# Autodesk Inventor assembly: Shooter Assembly
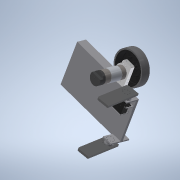
[picture p0: Inventor's stored thumbnail of the model, 180x180]
Saved by Autodesk Inventor 2021 (Build 250183000, 183)
## iProperties
Created: 2020-10-17
Part Number: Shooter Assembly
Document SubType Name: Assembly
Designer: Delta
Author: Delta
## Documents named in this file (9)
- C:\Robotics\CAD\2020-21-CAD\Shooter\Shooter Assembly.iam
- C:\Robotics\CAD\2020-21-CAD\Shooter\Guide.ipt
- C:\Robotics\CAD\2020-21-CAD\Shooter\Axle Rotate.ipt
- C:\Robotics\CAD\2020-21-CAD\Shooter\Triangle axle slide connector.ipt
- C:\Robotics\CAD\2020-21-CAD\Shooter\Tetrex 2pc motor mount.ipt
- C:\Robotics\CAD\2020-21-CAD\Shooter\motor-3102NeveRest20 (1).ipt
- C:\Robotics\CAD\2020-21-CAD\Shooter\Flywheel_4inWheel8mmHub.ipt
- C:\Robotics\CAD\2020-21-CAD\Shooter\Tetrix bracket - single servo.ipt
- C:\Robotics\CAD\COTSParts\Rev\REV-41-1097SmartServo.ipt
## Components (10 placed, 8 different names)
1. Guide:1 — Mate:14, Mate:15, Angle:1, Angle:2, Mate:37, Mate:38, Mate:39, Mate:40, Mate:43, Flush:8, Mate:44
2. Axle Rotate:1 — Mate:9, Mate:13, Mate:40
3. Axle Rotate:2 — Mate:8, Mate:12, Mate:37, Mate:38, Mate:39
4. Triangle axle slide connector:1 — Mate:8, Mate:12, Flush:9, Flush:10
5. Triangle axle slide connector:2 — Mate:9, Mate:13, Flush:9, Flush:10
6. Tetrex 2pc motor mount:1 — Mate:14, Mate:15, Angle:1, Mate:16, Mate:17
7. motor-3102NeveRest20 (1):1 — Mate:16, Mate:17, Mate:18, Mate:19, Angle:2
8. Flywheel_4inWheel8mmHub:1 — Mate:18, Mate:19
9. Tetrix bracket - single servo:1 — Mate:25, Mate:41, Mate:42, Mate:43, Flush:8
10. REV-41-1097SmartServo:1 — Mate:25, Mate:41, Mate:42, Mate:44
## Relationships (24: Mate 19, Flush 3, Angle 2)
- Mate:8: Axle Rotate:2 ↔ Triangle axle slide connector:1
- Mate:9: Axle Rotate:1 ↔ Triangle axle slide connector:2
- Mate:12: Axle Rotate:2 ↔ Triangle axle slide connector:1
- Mate:13: Axle Rotate:1 ↔ Triangle axle slide connector:2
- Mate:14: Guide:1 ↔ Tetrex 2pc motor mount:1
- Mate:15: Guide:1 ↔ Tetrex 2pc motor mount:1
- Angle:1 (0 deg): Guide:1 ↔ Tetrex 2pc motor mount:1
- Mate:16: Tetrex 2pc motor mount:1 ↔ motor-3102NeveRest20 (1):1
- Mate:17: Tetrex 2pc motor mount:1 ↔ motor-3102NeveRest20 (1):1
- Mate:18: motor-3102NeveRest20 (1):1 ↔ Flywheel_4inWheel8mmHub:1
- Mate:19: motor-3102NeveRest20 (1):1 ↔ Flywheel_4inWheel8mmHub:1
- Angle:2 (0 deg): Guide:1 ↔ motor-3102NeveRest20 (1):1
- Mate:25: Tetrix bracket - single servo:1 ↔ REV-41-1097SmartServo:1
- Mate:37: Guide:1 ↔ Axle Rotate:2
- Mate:38: Guide:1 ↔ Axle Rotate:2
- Mate:39: Guide:1 ↔ Axle Rotate:2
- Mate:40: Guide:1 ↔ Axle Rotate:1
- Mate:41: Tetrix bracket - single servo:1 ↔ REV-41-1097SmartServo:1
- Mate:42: Tetrix bracket - single servo:1 ↔ REV-41-1097SmartServo:1
- Mate:43: Guide:1 ↔ Tetrix bracket - single servo:1
- Flush:8: Guide:1 ↔ Tetrix bracket - single servo:1
- Mate:44: Guide:1 ↔ REV-41-1097SmartServo:1
- Flush:9: Triangle axle slide connector:1 ↔ Triangle axle slide connector:2
- Flush:10: Triangle axle slide connector:1 ↔ Triangle axle slide connector:2
